# Autodesk Inventor assembly: ASM_Micron_Open
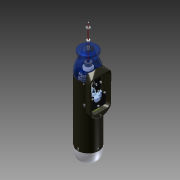
[picture p0: Inventor's stored thumbnail of the model, 180x180]
Saved by Autodesk Inventor 2011 SP2 (Build 150309200, 309)
## iProperties
Created: 2011-10-07
Part Number: ASM_Micron_Open
Document SubType Name: Assembly
Designer: sungwook
Author: sungwook
## Documents named in this file (14)
- C:\Users\sungwook\Documents\Inventor\Micron22_top_adj_02082013\Cannulation\ASM_Micron_Open.iam
- C:\Users\sungwook\Documents\Inventor\Micron22_top_adj_02082013\Assembly\Motion_Merge\Indep\ASM_Micron_ASAP_Indep0.iam
- C:\Users\sungwook\Documents\Inventor\Micron22_top_adj_02082013\Parts\ASAP\Handle_ASAP.iam
- C:\Users\sungwook\Documents\Inventor\Micron22_top_adj_02082013\Parts\Electronics\PCB_Stack.iam
- C:\Users\sungwook\Documents\Inventor\Micron22_top_adj_02082013\06082012_Outer_Tube\Outer_Tube.ipt
- C:\Users\sungwook\Documents\Inventor\Content Center Files\R2011\en-US\ANSI B18.6.3(00)\ANSI B18.6.3 - 0-80 UNF - 0.1875(32).ipt
- C:\Users\sungwook\Documents\Inventor\Micron22_top_adj_02082013\Parts\Handle\Ver2(Al_RP)\Handle_2_Back_rev2.ipt
- C:\Users\sungwook\Documents\Inventor\Micron22_top_adj_02082013\04192012_New_Front_2pcs\New_Front_Base_rev.ipt
- C:\Users\sungwook\Documents\Inventor\Micron22_top_adj_02082013\04192012_New_Front_2pcs\New_Front_Upper_rev_v2.ipt
- C:\Users\sungwook\Documents\Inventor\Micron22_top_adj_02082013\04192012_New_Front_2pcs\New_Front_Upper_rev_v3.ipt
- C:\Users\sungwook\Documents\Inventor\Micron22_top_adj_02082013\Parts\ASAP\Handle_ASAP2.iam
- C:\Users\sungwook\Documents\Inventor\Micron22_top_adj_02082013\Parts\ASAP\Handle_ASAP3.iam
- C:\Users\sungwook\Documents\Inventor\Micron22_top_adj_02082013\Cannulation\Cannulation_Asm.iam
- C:\Users\sungwook\Documents\Inventor\Micron22_top_adj_02082013\Cannulation\Cannulation_Asm_close.iam
## Components (15 placed, 13 different names)
1. (0,0,0) [sub-assembly] — Mate:2, Mate:73, Mate:74, Mate:107, Mate:108, Mate:55, Mate:139, Mate:142, Mate:143, Mate:144, Mate:145, Mate:146, Mate:147, Mate:148
2. Handle_ASAP:1 [sub-assembly] — Mate:55
3. PCB_Stack:1 [sub-assembly] — Flush:73, Mate:73, Mate:74
4. Handle_ASAP2:1 [sub-assembly] — Flush:127, Mate:139
5. Handle_ASAP3:1 [sub-assembly]
6. Cannulation_Asm_open [sub-assembly] — Mate:142, Mate:143, Mate:144, Mate:145
7. Cannulation_Asm_close:1 [sub-assembly] — Mate:146, Mate:147, Mate:148
8. New_Front_Base_rev:1 — Mate:112, Mate:113, Mate:114, Mate:120, Flush:121, Mate:121, Flush:123, Mate:141
9. New_Front_Upper_rev_v2:1 — Mate:120, Flush:121, Flush:122, Mate:138, Flush:128, Mate:140, Mate:141
10. New_Front_Upper_rev_v3:1 — Mate:121, Flush:123, Flush:124
11. Handle_2_Back_rev2:1 — Mate:109, Mate:110, Mate:111
12. Outer_Tube:1 — Mate:104, Mate:105, Mate:108, Mate:109, Mate:111, Mate:114, Flush:122, Flush:124, Mate:140
13. Cross Recessed 100° Flat Countersunk Head Machine Screw - Type I - Inch 0-80 UNF x 0.1875:1 — Mate:107
14. Cross Recessed 100° Flat Countersunk Head Machine Screw - Type I - Inch 0-80 UNF x 0.1875:2
15. Cross Recessed 100° Flat Countersunk Head Machine Screw - Type I - Inch 0-80 UNF x 0.1875:3
## Component patterns: (3 elements, first: Cross Recessed 100° Flat Countersunk Head Machine Screw - Type I - Inch 0-80 UNF x 0.1875:1)
## Relationships (35: Mate 27, Flush 8)
- Mate:2: (0,0,0)
- Mate:55: (0,0,0) ↔ Handle_ASAP:1
- Flush:73: PCB_Stack:1
- Mate:73: (0,0,0) ↔ PCB_Stack:1
- Mate:74: (0,0,0) ↔ PCB_Stack:1
- Mate:104: Outer_Tube:1
- Mate:105: Outer_Tube:1
- Mate:108: (0,0,0) ↔ Outer_Tube:1
- Mate:109: Handle_2_Back_rev2:1 ↔ Outer_Tube:1
- Mate:110: Handle_2_Back_rev2:1
- Mate:111: Handle_2_Back_rev2:1 ↔ Outer_Tube:1
- Mate:112: New_Front_Base_rev:1
- Mate:113: New_Front_Base_rev:1
- Mate:114: New_Front_Base_rev:1 ↔ Outer_Tube:1
- Mate:120: New_Front_Base_rev:1 ↔ New_Front_Upper_rev_v2:1
- Flush:121: New_Front_Base_rev:1 ↔ New_Front_Upper_rev_v2:1
- Flush:122: New_Front_Upper_rev_v2:1 ↔ Outer_Tube:1
- Mate:121: New_Front_Base_rev:1 ↔ New_Front_Upper_rev_v3:1
- Flush:123: New_Front_Base_rev:1 ↔ New_Front_Upper_rev_v3:1
- Flush:124: New_Front_Upper_rev_v3:1 ↔ Outer_Tube:1
- Flush:126 (24.5 mm)
- Flush:127: Handle_ASAP2:1
- Mate:138: New_Front_Upper_rev_v2:1
- Flush:128: New_Front_Upper_rev_v2:1
- Mate:139: (0,0,0) ↔ Handle_ASAP2:1
- Mate:140: New_Front_Upper_rev_v2:1 ↔ Outer_Tube:1
- Mate:141: New_Front_Base_rev:1 ↔ New_Front_Upper_rev_v2:1
- Mate:142: (0,0,0) ↔ Cannulation_Asm_open
- Mate:143: (0,0,0) ↔ Cannulation_Asm_open
- Mate:144: (0,0,0) ↔ Cannulation_Asm_open
- Mate:145: (0,0,0) ↔ Cannulation_Asm_open
- Mate:146: (0,0,0) ↔ Cannulation_Asm_close:1
- Mate:147: (0,0,0) ↔ Cannulation_Asm_close:1
- Mate:148: (0,0,0) ↔ Cannulation_Asm_close:1
- Mate:107: (0,0,0) ↔ Cross Recessed 100° Flat Countersunk Head Machine Screw - Type I - Inch 0-80 UNF x 0.1875:1
